# Autodesk Inventor assembly: 2019 DRIVEBASE IDEAS
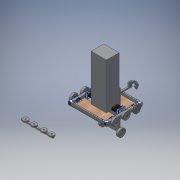
[picture p0: Inventor's stored thumbnail of the model, 180x180]
Saved by Autodesk Inventor 2018 (Build 220112000, 112)
## iProperties
Created: 2018-11-23
Part Number: 2019 DRIVEBASE IDEAS
Document SubType Name: Assembly
Designer: maste
Sending System: Autodesk Inventor 2019
Preprocessor: ST-DEVELOPER v17
Title: D:\Summer Drive Base V1\Summer Drivebase\Practice Drivebase Assembly.stp
Author: maste
## Documents named in this file (17)
- C:\Users\Gabriel\Documents\GitHub\2019CAD\Summer Drivebase\2019 DRIVEBASE IDEAS.iam
- C:\Users\Gabriel\Documents\GitHub\2019CAD\Summer Drivebase\Drive Tube Assem.iam
- C:\Users\Gabriel\Documents\GitHub\2019CAD\Summer Drivebase\6in Colson Assem.iam
- C:\Users\Gabriel\Documents\GitHub\2019CAD\Summer Drivebase\Omni Wheel.iam
- C:\Users\Gabriel\Documents\GitHub\2019CAD\Summer Drivebase\Bumper Assem Full.iam
- C:\Users\Gabriel\Documents\GitHub\2019CAD\Summer Drivebase\0.125in Spacer.ipt
- C:\Users\Gabriel\Documents\GitHub\2019CAD\Summer Drivebase\Belly Pan V2.ipt
- C:\Users\Gabriel\Documents\GitHub\2019CAD\Summer Drivebase\26in 2x1.ipt
- C:\Users\Gabriel\Documents\GitHub\2019CAD\Summer Drivebase\Sax Gusset.ipt
- C:\Users\Gabriel\Documents\GitHub\2019CAD\ElevatorRep.ipt
- C:\Users\Gabriel\Documents\GitHub\2019CAD\RobotStilts.ipt
- C:\Users\Gabriel\Documents\GitHub\2019CAD\HatchArm.ipt
- C:\Users\Gabriel\Documents\GitHub\2019CAD\HatchArmGripper.ipt
- C:\Users\Gabriel\Documents\GitHub\2019CAD\HatchArmGripperFingers.ipt
- C:\Users\Gabriel\Documents\GitHub\2019CAD\Arrow.ipt
- C:\Users\Gabriel\Documents\GitHub\2019CAD\VacuumWheels.ipt
- C:\Users\Gabriel\Documents\GitHub\2019CAD\VacuumBar.ipt
## Components (35 placed, 16 different names)
1. Drive Tube Assem:1 [sub-assembly] — Mate:40, Mate:46, Mate:47, Mate:48, Mate:49, Mate:50, Mate:52, Mate:53, Mate:54, Mate:55, Mate:56, Mate:57, Mate:58, Mate:68, Mate:69, Mate:70, Mate:86, Mate:87, Mate:88, Mate:92, Mate:93, Mate:94
2. Drive Tube Assem:2 [sub-assembly] — Mate:31, Mate:32, Mate:39, Mate:41, Mate:43, Mate:44, Mate:45, Mate:59, Mate:60, Mate:61, Mate:62, Mate:63, Mate:64, Mate:65, Mate:66, Mate:67, Mate:77, Mate:78, Mate:79, Mate:98, Mate:99, Mate:100
3. 6in Colson Assem:1 [sub-assembly] — Mate:56, Mate:57, Mate:58
4. 6in Colson Assem:2 [sub-assembly] — Mate:52, Mate:53, Mate:54, Mate:55
5. 6in Colson Assem:3 [sub-assembly] — Mate:62, Mate:63, Mate:64
6. 6in Colson Assem:4 [sub-assembly] — Mate:59, Mate:60, Mate:61
7. Omni Wheel:1 [sub-assembly] — Mate:31, Mate:32, Mate:42
8. Omni Wheel:2 [sub-assembly] — Mate:49, Mate:50, Mate:51
9. Bumper Assem Full:1 [sub-assembly] — Mate:39, Mate:40, Mate:41
10. 0.125in Spacer:1 — Mate:42, Mate:43, Mate:44, Mate:45
11. 0.125in Spacer:2 — Mate:46, Mate:47, Mate:48, Mate:51
12. Belly Pan V2:1 — Mate:65, Mate:66, Mate:67, Mate:68, Mate:69, Mate:70, Mate:71, Mate:72, Mate:73, Mate:74, Mate:75, Mate:76, Mate:80, Mate:81, Mate:82, Mate:83, Mate:84, Mate:85, Mate:89, Mate:90, Mate:91, Mate:95, Mate:96, Mate:97, Mate:101, Mate:102
13. 26in 2x1:1 — Mate:74, Mate:75, Mate:76
14. 26in 2x1:2 — Mate:71, Mate:72, Mate:73
15. Sax Gusset:1 — Mate:77, Mate:78, Mate:79
16. Sax Gusset:2 — Mate:80, Mate:81, Mate:82
17. Sax Gusset:3 — Mate:92, Mate:93, Mate:94
18. Sax Gusset:4 — Mate:89, Mate:90, Mate:91
19. Sax Gusset:5 — Mate:95, Mate:96, Mate:97
20. Sax Gusset:6 — Mate:98, Mate:99, Mate:100
21. Sax Gusset:7 — Mate:83, Mate:84, Mate:85
22. Sax Gusset:8 — Mate:86, Mate:87, Mate:88
23. ElevatorRep:1 — Mate:101, Mate:102, Mate:103, Mate:104
24. RobotStilts:1 — Mate:103, Mate:104, Mate:119, Mate:120
25. HatchArm:1 — Mate:105, Mate:106, Mate:107, Mate:108, Mate:109, Mate:110, Mate:111
26. HatchArmGripperThumb:1 — Mate:105, Mate:106, Mate:107
27. HatchArmGripperFingers:1 — Mate:108, Mate:109, Mate:110, Mate:111, Mate:112, Mate:113, Mate:114
28. Arrow:1 — Mate:112, Mate:113, Mate:114
29. VacuumWheels:1 — Mate:118
30. VacuumBar:1 — Mate:115, Mate:116, Mate:117, Mate:118
31. VacuumWheels:2 — Mate:117
32. VacuumWheels:3 — Mate:116
33. VacuumWheels:4 — Mate:115
34. 6in Colson Assem:5 [sub-assembly] — Mate:119
35. 6in Colson Assem:6 [sub-assembly] — Mate:120
## Relationships (84: Mate 84)
- Mate:31: Drive Tube Assem:2 ↔ Omni Wheel:1
- Mate:32: Drive Tube Assem:2 ↔ Omni Wheel:1
- Mate:39: Drive Tube Assem:2 ↔ Bumper Assem Full:1
- Mate:40: Drive Tube Assem:1 ↔ Bumper Assem Full:1
- Mate:41: Drive Tube Assem:2 ↔ Bumper Assem Full:1
- Mate:42: Omni Wheel:1 ↔ 0.125in Spacer:1
- Mate:43: Drive Tube Assem:2 ↔ 0.125in Spacer:1
- Mate:44: Drive Tube Assem:2 ↔ 0.125in Spacer:1
- Mate:45: Drive Tube Assem:2 ↔ 0.125in Spacer:1
- Mate:46: Drive Tube Assem:1 ↔ 0.125in Spacer:2
- Mate:47: Drive Tube Assem:1 ↔ 0.125in Spacer:2
- Mate:48: Drive Tube Assem:1 ↔ 0.125in Spacer:2
- Mate:49: Drive Tube Assem:1 ↔ Omni Wheel:2
- Mate:50: Drive Tube Assem:1 ↔ Omni Wheel:2
- Mate:51: Omni Wheel:2 ↔ 0.125in Spacer:2
- Mate:52: Drive Tube Assem:1 ↔ 6in Colson Assem:2
- Mate:53: Drive Tube Assem:1 ↔ 6in Colson Assem:2
- Mate:54: Drive Tube Assem:1 ↔ 6in Colson Assem:2
- Mate:55: Drive Tube Assem:1 ↔ 6in Colson Assem:2
- Mate:56: Drive Tube Assem:1 ↔ 6in Colson Assem:1
- Mate:57: Drive Tube Assem:1 ↔ 6in Colson Assem:1
- Mate:58: Drive Tube Assem:1 ↔ 6in Colson Assem:1
- Mate:59: Drive Tube Assem:2 ↔ 6in Colson Assem:4
- Mate:60: Drive Tube Assem:2 ↔ 6in Colson Assem:4
- Mate:61: Drive Tube Assem:2 ↔ 6in Colson Assem:4
- Mate:62: Drive Tube Assem:2 ↔ 6in Colson Assem:3
- Mate:63: Drive Tube Assem:2 ↔ 6in Colson Assem:3
- Mate:64: Drive Tube Assem:2 ↔ 6in Colson Assem:3
- Mate:65: Drive Tube Assem:2 ↔ Belly Pan V2:1
- Mate:66: Drive Tube Assem:2 ↔ Belly Pan V2:1
- Mate:67: Drive Tube Assem:2 ↔ Belly Pan V2:1
- Mate:68: Drive Tube Assem:1 ↔ Belly Pan V2:1
- Mate:69: Drive Tube Assem:1 ↔ Belly Pan V2:1
- Mate:70: Drive Tube Assem:1 ↔ Belly Pan V2:1
- Mate:71: Belly Pan V2:1 ↔ 26in 2x1:2
- Mate:72: Belly Pan V2:1 ↔ 26in 2x1:2
- Mate:73: Belly Pan V2:1 ↔ 26in 2x1:2
- Mate:74: Belly Pan V2:1 ↔ 26in 2x1:1
- Mate:75: Belly Pan V2:1 ↔ 26in 2x1:1
- Mate:76: Belly Pan V2:1 ↔ 26in 2x1:1
- Mate:77: Drive Tube Assem:2 ↔ Sax Gusset:1
- Mate:78: Drive Tube Assem:2 ↔ Sax Gusset:1
- Mate:79: Drive Tube Assem:2 ↔ Sax Gusset:1
- Mate:80: Belly Pan V2:1 ↔ Sax Gusset:2
- Mate:81: Belly Pan V2:1 ↔ Sax Gusset:2
- Mate:82: Belly Pan V2:1 ↔ Sax Gusset:2
- Mate:83: Belly Pan V2:1 ↔ Sax Gusset:7
- Mate:84: Belly Pan V2:1 ↔ Sax Gusset:7
- Mate:85: Belly Pan V2:1 ↔ Sax Gusset:7
- Mate:86: Drive Tube Assem:1 ↔ Sax Gusset:8
- Mate:87: Drive Tube Assem:1 ↔ Sax Gusset:8
- Mate:88: Drive Tube Assem:1 ↔ Sax Gusset:8
- Mate:89: Belly Pan V2:1 ↔ Sax Gusset:4
- Mate:90: Belly Pan V2:1 ↔ Sax Gusset:4
- Mate:91: Belly Pan V2:1 ↔ Sax Gusset:4
- Mate:92: Drive Tube Assem:1 ↔ Sax Gusset:3
- Mate:93: Drive Tube Assem:1 ↔ Sax Gusset:3
- Mate:94: Drive Tube Assem:1 ↔ Sax Gusset:3
- Mate:95: Belly Pan V2:1 ↔ Sax Gusset:5
- Mate:96: Belly Pan V2:1 ↔ Sax Gusset:5
- Mate:97: Belly Pan V2:1 ↔ Sax Gusset:5
- Mate:98: Drive Tube Assem:2 ↔ Sax Gusset:6
- Mate:99: Drive Tube Assem:2 ↔ Sax Gusset:6
- Mate:100: Drive Tube Assem:2 ↔ Sax Gusset:6
- Mate:101: Belly Pan V2:1 ↔ ElevatorRep:1
- Mate:102: Belly Pan V2:1 ↔ ElevatorRep:1
- Mate:103: ElevatorRep:1 ↔ RobotStilts:1
- Mate:104: ElevatorRep:1 ↔ RobotStilts:1
- Mate:105: HatchArm:1 ↔ HatchArmGripperThumb:1
- Mate:106: HatchArm:1 ↔ HatchArmGripperThumb:1
- Mate:107: HatchArm:1 ↔ HatchArmGripperThumb:1
- Mate:108: HatchArm:1 ↔ HatchArmGripperFingers:1
- Mate:109: HatchArm:1 ↔ HatchArmGripperFingers:1
- Mate:110: HatchArm:1 ↔ HatchArmGripperFingers:1
- Mate:111: HatchArm:1 ↔ HatchArmGripperFingers:1
- Mate:112: HatchArmGripperFingers:1 ↔ Arrow:1
- Mate:113: HatchArmGripperFingers:1 ↔ Arrow:1
- Mate:114: HatchArmGripperFingers:1 ↔ Arrow:1
- Mate:115: VacuumBar:1 ↔ VacuumWheels:4
- Mate:116: VacuumBar:1 ↔ VacuumWheels:3
- Mate:117: VacuumBar:1 ↔ VacuumWheels:2
- Mate:118: VacuumWheels:1 ↔ VacuumBar:1
- Mate:119: RobotStilts:1 ↔ 6in Colson Assem:5
- Mate:120: RobotStilts:1 ↔ 6in Colson Assem:6
